# Autodesk Inventor assembly: linac
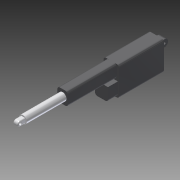
[picture p0: Inventor's stored thumbnail of the model, 180x180]
Saved by Autodesk Inventor 2011 (Build 150239000, 239)
## iProperties
Created: 2011-10-08
Part Number: linac
Document SubType Name: Assembly
Designer: Matthew
Author: Matthew
## Documents named in this file (3)
- C:\Users\Matthew\Documents\matthew_autocad\prlite\arm perhaps\linac.iam
- C:\Users\Matthew\Documents\matthew_autocad\prlite\arm perhaps\linac body.ipt
- C:\Users\Matthew\Documents\matthew_autocad\prlite\arm perhaps\linac arm1.ipt
## Components (2 placed, 2 different names)
1. linac body:1 — Mate:4, Flush:1, Flush:2
2. linac arm1:1 — Mate:4, Flush:1, Flush:2
## Relationships (3: Flush 2, Mate 1)
- Mate:4: linac body:1 ↔ linac arm1:1
- Flush:1 (10.287 mm): linac body:1 ↔ linac arm1:1
- Flush:2: linac body:1 ↔ linac arm1:1
